# Autodesk Inventor assembly: CRA-ASM-1002
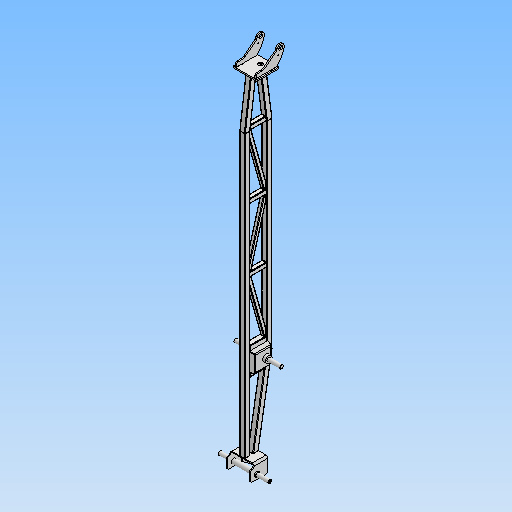
[picture p0: Inventor's stored thumbnail of the model, 512x512]
Saved by Autodesk Inventor 2025.4 (Build 294407000, 407)
## iProperties
Created: 2025-12-20
Part Number: CRA-ASM-1002
Document SubType Name: Assembly
Designer: josh
Description: CLEANING ROBOT ARM WELDMENT
Mass: 22137.9 g
Surface Area: 20106.2 cm^2
Volume: 2820.11 cm^3
Density: 7.85 g/cm^3
Author: josh
## Documents named in this file (23)
- R:\A1- Neuweg Design Data\OM Robotics\CLEANING ROBOT TOWER PROJECT\CRA-ASM-1002.iam
- R:\A1- Neuweg Design Data\OM Robotics\CLEANING ROBOT TOWER PROJECT\CRA-1002.ipt
- R:\A1- Neuweg Design Data\OM Robotics\CLEANING ROBOT TOWER PROJECT\CRA-1003.ipt
- R:\A1- Neuweg Design Data\OM Robotics\CLEANING ROBOT TOWER PROJECT\CRA-1004.ipt
- R:\A1- Neuweg Design Data\OM Robotics\CLEANING ROBOT TOWER PROJECT\CRA-1005.ipt
- R:\A1- Neuweg Design Data\OM Robotics\CLEANING ROBOT TOWER PROJECT\CRA-1006.ipt
- R:\A1- Neuweg Design Data\OM Robotics\CLEANING ROBOT TOWER PROJECT\CRA-1007.ipt
- R:\A1- Neuweg Design Data\OM Robotics\CLEANING ROBOT TOWER PROJECT\CRA-1008.ipt
- R:\A1- Neuweg Design Data\OM Robotics\CLEANING ROBOT TOWER PROJECT\CRA-1009.ipt
- R:\A1- Neuweg Design Data\OM Robotics\CLEANING ROBOT TOWER PROJECT\CRA-1010.ipt
- R:\A1- Neuweg Design Data\OM Robotics\CLEANING ROBOT TOWER PROJECT\CRA-1011.ipt
- R:\A1- Neuweg Design Data\OM Robotics\CLEANING ROBOT TOWER PROJECT\CRA-1012.ipt
- R:\A1- Neuweg Design Data\OM Robotics\CLEANING ROBOT TOWER PROJECT\CRA-1013.ipt
- R:\A1- Neuweg Design Data\OM Robotics\CLEANING ROBOT TOWER PROJECT\CRA-1014.ipt
- R:\A1- Neuweg Design Data\OM Robotics\CLEANING ROBOT TOWER PROJECT\CRA-1015.ipt
- R:\A1- Neuweg Design Data\OM Robotics\CLEANING ROBOT TOWER PROJECT\CRA-1016.ipt
- R:\A1- Neuweg Design Data\OM Robotics\CLEANING ROBOT TOWER PROJECT\CRA-1017.ipt
- R:\A1- Neuweg Design Data\OM Robotics\CLEANING ROBOT TOWER PROJECT\CRA-1018.ipt
- R:\A1- Neuweg Design Data\OM Robotics\CLEANING ROBOT TOWER PROJECT\CRA-1019.ipt
- R:\A1- Neuweg Design Data\OM Robotics\CLEANING ROBOT TOWER PROJECT\CRA-1020.ipt
- R:\A1- Neuweg Design Data\OM Robotics\CLEANING ROBOT TOWER PROJECT\CRA-1021.ipt
- R:\A1- Neuweg Design Data\OM Robotics\CLEANING ROBOT TOWER PROJECT\CRA-1023.ipt
- R:\A1- Neuweg Design Data\OM Robotics\CLEANING ROBOT TOWER PROJECT\CRA-1024.ipt
## Components (24 placed, 22 different names)
1. CRA-1002:1
2. CRA-1003:1
3. CRA-1004:1
4. CRA-1005:1
5. CRA-1006:1
6. CRA-1007:1
7. CRA-1008:1
8. CRA-1009:1
9. CRA-1010:1
10. CRA-1011:1
11. CRA-1012:1
12. CRA-1013:1
13. CRA-1014:1
14. CRA-1015:1
15. CRA-1016:1
16. CRA-1017:1
17. CRA-1018:1
18. CRA-1019:1 — Insert:1
19. CRA-1020:1
20. CRA-1021:1
21. CRA-1023:1
22. CRA-1024:1
23. CRA-1016:3 — Flush:4, Flush:3, Flush:1
24. CRA-1020:2 — Insert:1
## Relationships (4: Flush 3, Insert 1)
- Flush:4 (-136.525 mm): CRA-1016:3
- Flush:3: CRA-1016:3
- Flush:1: CRA-1016:3
- Insert:1: CRA-1019:1 ↔ CRA-1020:2
